# Autodesk Inventor assembly: RCR_drive
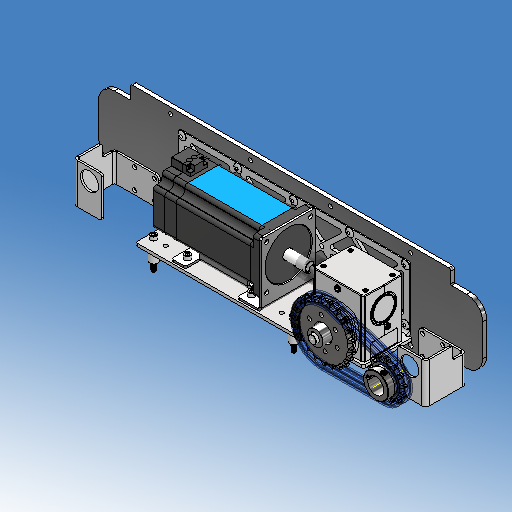
[picture p0: Inventor's stored thumbnail of the model, 512x512]
Saved by Autodesk Inventor 2025 (Build 290162000, 162)
## iProperties
Created: 2024-02-27
Part Number: RCR_drive
Document SubType Name: Assembly
Designer: seene
Author: seene
## Documents named in this file (21)
- C:\Users\seene\Desktop\Stony Brook\SBRT\RCR_Dexter\Drive\RCR_drive.iam
- C:\Users\seene\Desktop\Stony Brook\SBRT\RCR_Dexter\Drive\v1\ChassisInterface.ipt
- C:\Users\seene\Desktop\Stony Brook\SBRT\RCR_Dexter\Drive\v1\2299K28_Flat Sprocket.ipt
- C:\Users\seene\Desktop\Stony Brook\SBRT\RCR_Dexter\Drive\v1\5887K172_Right-Angle Speed Reducer.ipt
- C:\Users\seene\Desktop\Stony Brook\SBRT\RCR_Dexter\Drive\v1\9939T12_Durometer 64D Spider for 1-5 16 OD Set Screw Vibrate-Damping Precision Flexible Shaft Coupling.ipt
- C:\Users\seene\Desktop\Stony Brook\SBRT\RCR_Dexter\Drive\v1\9939T102_Vibrate-Damping Precision Flexible Shaft Coupling.ipt
- C:\Users\seene\Desktop\Stony Brook\SBRT\RCR_Dexter\Drive\v1\9939T104_Vibrate-Damping Precision Flexible Shaft Coupling.ipt
- C:\Users\seene\Desktop\Stony Brook\SBRT\RCR_Dexter\Drive\v1\am-0077a 500 Key Hub REV3.ipt
- C:\Users\seene\Desktop\Stony Brook\SBRT\RCR_Dexter\Drive\v1\6280K675_Roller Chain Sprocket.ipt
- C:\Users\seene\Desktop\Stony Brook\SBRT\RCR_Dexter\Drive\QuintinCAD\NEMA34_gearbox_sheetMetaMount.ipt
- C:\Users\seene\Desktop\Stony Brook\SBRT\RCR_Dexter\Drive\v1\40 chain link.ipt
- C:\Users\seene\Desktop\Stony Brook\SBRT\RCR_Dexter\Drive\v1\34HS59-6004D-E1000 .ipt
- C:\Users\seene\Desktop\Stony Brook\SBRT\RCR_Dexter\Drive\v1\VTR-037_pulley.ipt
- C:\Users\seene\Desktop\Stony Brook\SBRT\RCR_Dexter\Drive\v1\StepperMotorStandOff.ipt
- C:\Users\seene\Desktop\Stony Brook\SBRT\RCR_Dexter\Drive\v1\DriveShaftSupport.ipt
- C:\Users\seene\Desktop\Stony Brook\SBRT\RCR_Dexter\Drive\v1\DriveShaftSupport _Flipped.ipt
- C:\Users\seene\Desktop\Stony Brook\SBRT\RCR_Dexter\Drive\RCR_drive\Design Accelerator\Chain Drive3.iam
- C:\Users\seene\Desktop\Stony Brook\SBRT\RCR_Dexter\Drive\v1\90128A252_Zinc-Plated Alloy Steel Socket Head Screw.ipt
- C:\Users\seene\Desktop\Stony Brook\SBRT\RCR_Dexter\Drive\v1\DriveMountStandoff.ipt
- C:\Users\seene\Desktop\Stony Brook\SBRT\RCR_Dexter\Drive\v1\91274A156_Zinc-Aluminum-Coated Alloy Steel Socket Head Screw.ipt
- C:\Users\seene\Desktop\Stony Brook\SBRT\RCR_Dexter\Drive\v1\97525A550_18-8 Stainless Steel Blind Rivets.ipt
## Components (41 placed, 20 different names)
1. 2299K28_Flat Sprocket:1 — Mate:23, Mate:24, Mate:25, Flush:7, Mate:133, Mate:134, Mate:135, Mate:136, Mate:137, Flush:29
2. 5887K172_Right-Angle Speed Reducer:1 — Mate:5, Mate:6, Mate:26, Mate:66, Mate:67, Mate:68, Mate:162
3. 9939T12_Durometer 64D Spider for 1-5 16 OD Set Screw Vibrate-Damping Precision Flexible Shaft Coupling:1 — Mate:1, Mate:7, Mate:8, Mate:9
4. 9939T102_Vibrate-Damping Precision Flexible Shaft Coupling:1 — Mate:5, Mate:6, Mate:8, Mate:9
5. 9939T104_Vibrate-Damping Precision Flexible Shaft Coupling:1 — Mate:1, Mate:7
6. am-0077a 500 Key Hub REV3:1 — Mate:23, Mate:24, Mate:25, Mate:26, Mate:162
7. 6280K675_Roller Chain Sprocket:1 — Flush:7, Mate:312
8. NEMA34_gearbox_sheetMetaMount:1 — Mate:66, Mate:67, Mate:68, Mate:167, Mate:249, Mate:250, Mate:254, Mate:258, Mate:259, Mate:313, Mate:314, Mate:316, Mate:319, Mate:320
9. 34HS59-6004D-E1000 :1 — Mate:251, Flush:45, Mate:255, Mate:256, Mate:257
10. ChassisInterface:2 — Mate:167, Mate:249, Mate:250, Mate:281, Mate:282, Mate:287, Mate:309, Mate:310, Mate:311
11. VTR-037_pulley:1
12. StepperMotorStandOff:1 — Mate:251, Flush:45, Mate:254, Mate:255, Mate:256, Mate:257, Mate:258, Mate:259, Mate:317, Mate:318
13. DriveShaftSupport:1 — Mate:281, Mate:282, Mate:287
14. DriveShaftSupport _Flipped:1 — Mate:309, Mate:310, Mate:311, Mate:312
15. Chain Drive:2 [sub-assembly]
16. 40 chain link:1 — Mate:127, Mate:130, Mate:136, Mate:137
17. 40 chain link:2 — Mate:129, Mate:132, Mate:135, Flush:29
18. 40 chain link:3 — Mate:128, Mate:129, Mate:131, Mate:132, Mate:134
19. 40 chain link:4 — Mate:127, Mate:128, Mate:130, Mate:131, Mate:133
20. 90128A252_Zinc-Plated Alloy Steel Socket Head Screw:1 — Mate:315, Mate:316
21. DriveMountStandoff:1 — Mate:313, Mate:314, Mate:315
22. 90128A252_Zinc-Plated Alloy Steel Socket Head Screw:2
23. DriveMountStandoff:2
24. 90128A252_Zinc-Plated Alloy Steel Socket Head Screw:3
25. DriveMountStandoff:3
26. 90128A252_Zinc-Plated Alloy Steel Socket Head Screw:4
27. DriveMountStandoff:4
28. 91274A156_Zinc-Aluminum-Coated Alloy Steel Socket Head Screw:1 — Mate:317, Mate:318
29. 91274A156_Zinc-Aluminum-Coated Alloy Steel Socket Head Screw:2
30. 91274A156_Zinc-Aluminum-Coated Alloy Steel Socket Head Screw:3
31. 91274A156_Zinc-Aluminum-Coated Alloy Steel Socket Head Screw:4
32. 97525A550_18-8 Stainless Steel Blind Rivets:1 — Mate:319, Mate:320
33. 97525A550_18-8 Stainless Steel Blind Rivets:2
34. 97525A550_18-8 Stainless Steel Blind Rivets:3
35. 97525A550_18-8 Stainless Steel Blind Rivets:4
36. 97525A550_18-8 Stainless Steel Blind Rivets:5
37. 97525A550_18-8 Stainless Steel Blind Rivets:6
38. 97525A550_18-8 Stainless Steel Blind Rivets:7
39. 97525A550_18-8 Stainless Steel Blind Rivets:8
40. 97525A550_18-8 Stainless Steel Blind Rivets:9
41. 97525A550_18-8 Stainless Steel Blind Rivets:10
## Component patterns: (4 elements, first: 90128A252_Zinc-Plated Alloy Steel Socket Head Screw:1 + DriveMountStandoff:1), (4 elements, first: 91274A156_Zinc-Aluminum-Coated Alloy Steel Socket Head Screw:1), (10 elements, first: 97525A550_18-8 Stainless Steel Blind Rivets:1)
## Relationships (53: Mate 50, Flush 3)
- Mate:1: 9939T12_Durometer 64D Spider for 1-5 16 OD Set Screw Vibrate-Damping Precision Flexible Shaft Coupling:1 ↔ 9939T104_Vibrate-Damping Precision Flexible Shaft Coupling:1
- Mate:5 (9.525 mm): 5887K172_Right-Angle Speed Reducer:1 ↔ 9939T102_Vibrate-Damping Precision Flexible Shaft Coupling:1
- Mate:6: 5887K172_Right-Angle Speed Reducer:1 ↔ 9939T102_Vibrate-Damping Precision Flexible Shaft Coupling:1
- Mate:7: 9939T12_Durometer 64D Spider for 1-5 16 OD Set Screw Vibrate-Damping Precision Flexible Shaft Coupling:1 ↔ 9939T104_Vibrate-Damping Precision Flexible Shaft Coupling:1
- Mate:8: 9939T12_Durometer 64D Spider for 1-5 16 OD Set Screw Vibrate-Damping Precision Flexible Shaft Coupling:1 ↔ 9939T102_Vibrate-Damping Precision Flexible Shaft Coupling:1
- Mate:9: 9939T12_Durometer 64D Spider for 1-5 16 OD Set Screw Vibrate-Damping Precision Flexible Shaft Coupling:1 ↔ 9939T102_Vibrate-Damping Precision Flexible Shaft Coupling:1
- Mate:23: 2299K28_Flat Sprocket:1 ↔ am-0077a 500 Key Hub REV3:1
- Mate:24: 2299K28_Flat Sprocket:1 ↔ am-0077a 500 Key Hub REV3:1
- Mate:25: 2299K28_Flat Sprocket:1 ↔ am-0077a 500 Key Hub REV3:1
- Mate:26: 5887K172_Right-Angle Speed Reducer:1 ↔ am-0077a 500 Key Hub REV3:1
- Flush:7: 2299K28_Flat Sprocket:1 ↔ 6280K675_Roller Chain Sprocket:1
- Mate:66: 5887K172_Right-Angle Speed Reducer:1 ↔ NEMA34_gearbox_sheetMetaMount:1
- Mate:67: 5887K172_Right-Angle Speed Reducer:1 ↔ NEMA34_gearbox_sheetMetaMount:1
- Mate:68: 5887K172_Right-Angle Speed Reducer:1 ↔ NEMA34_gearbox_sheetMetaMount:1
- Mate:127: 40 chain link:1 ↔ 40 chain link:4
- Mate:128: 40 chain link:3 ↔ 40 chain link:4
- Mate:129: 40 chain link:2 ↔ 40 chain link:3
- Mate:130: 40 chain link:1 ↔ 40 chain link:4
- Mate:131: 40 chain link:3 ↔ 40 chain link:4
- Mate:132: 40 chain link:2 ↔ 40 chain link:3
- Mate:133: 2299K28_Flat Sprocket:1 ↔ 40 chain link:4
- Mate:134: 2299K28_Flat Sprocket:1 ↔ 40 chain link:3
- Mate:135: 2299K28_Flat Sprocket:1 ↔ 40 chain link:2
- Mate:136: 2299K28_Flat Sprocket:1 ↔ 40 chain link:1
- Mate:137: 2299K28_Flat Sprocket:1 ↔ 40 chain link:1
- Flush:29 (-3.175 mm): 2299K28_Flat Sprocket:1 ↔ 40 chain link:2
- Mate:162 (1.5875 mm): 5887K172_Right-Angle Speed Reducer:1 ↔ am-0077a 500 Key Hub REV3:1
- Mate:167: NEMA34_gearbox_sheetMetaMount:1 ↔ ChassisInterface:2
- Mate:249: NEMA34_gearbox_sheetMetaMount:1 ↔ ChassisInterface:2
- Mate:250: NEMA34_gearbox_sheetMetaMount:1 ↔ ChassisInterface:2
- Mate:251: 34HS59-6004D-E1000 :1 ↔ StepperMotorStandOff:1
- Flush:45: 34HS59-6004D-E1000 :1 ↔ StepperMotorStandOff:1
- Mate:254: NEMA34_gearbox_sheetMetaMount:1 ↔ StepperMotorStandOff:1
- Mate:255: 34HS59-6004D-E1000 :1 ↔ StepperMotorStandOff:1
- Mate:256: 34HS59-6004D-E1000 :1 ↔ StepperMotorStandOff:1
- Mate:257: 34HS59-6004D-E1000 :1 ↔ StepperMotorStandOff:1
- Mate:258: NEMA34_gearbox_sheetMetaMount:1 ↔ StepperMotorStandOff:1
- Mate:259: NEMA34_gearbox_sheetMetaMount:1 ↔ StepperMotorStandOff:1
- Mate:281: ChassisInterface:2 ↔ DriveShaftSupport:1
- Mate:282: ChassisInterface:2 ↔ DriveShaftSupport:1
- Mate:287: ChassisInterface:2 ↔ DriveShaftSupport:1
- Mate:309: ChassisInterface:2 ↔ DriveShaftSupport _Flipped:1
- Mate:310: ChassisInterface:2 ↔ DriveShaftSupport _Flipped:1
- Mate:311: ChassisInterface:2 ↔ DriveShaftSupport _Flipped:1
- Mate:312: 6280K675_Roller Chain Sprocket:1 ↔ DriveShaftSupport _Flipped:1
- Mate:313: NEMA34_gearbox_sheetMetaMount:1 ↔ DriveMountStandoff:1
- Mate:314: NEMA34_gearbox_sheetMetaMount:1 ↔ DriveMountStandoff:1
- Mate:315: 90128A252_Zinc-Plated Alloy Steel Socket Head Screw:1 ↔ DriveMountStandoff:1
- Mate:316: NEMA34_gearbox_sheetMetaMount:1 ↔ 90128A252_Zinc-Plated Alloy Steel Socket Head Screw:1
- Mate:317: StepperMotorStandOff:1 ↔ 91274A156_Zinc-Aluminum-Coated Alloy Steel Socket Head Screw:1
- Mate:318: StepperMotorStandOff:1 ↔ 91274A156_Zinc-Aluminum-Coated Alloy Steel Socket Head Screw:1
- Mate:319: NEMA34_gearbox_sheetMetaMount:1 ↔ 97525A550_18-8 Stainless Steel Blind Rivets:1
- Mate:320: NEMA34_gearbox_sheetMetaMount:1 ↔ 97525A550_18-8 Stainless Steel Blind Rivets:1
